# Autodesk Inventor assembly: 2021-2022 Wheel Module
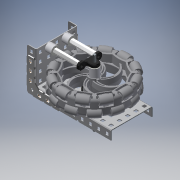
[picture p0: Inventor's stored thumbnail of the model, 180x180]
Saved by Autodesk Inventor 2019 (Build 230136000, 136)
## iProperties
Created: 2021-08-26
Part Number: 2021-2022 Wheel Module
Document SubType Name: Assembly
Designer: 22spencen
Author: 22spencen
## Documents named in this file (13)
- \\Chopper\2022\22spencen\Documents\VEX_CAD\Assemblies\2021-2022 Wheel Module.iam
- U:\Svec\Robotics\Parts\Motion\4_Omni-Directional_Wheel_276-2185.ipt
- U:\Svec\Robotics\Parts\Motion\Metal_Shaft_Inserts_276-3881-002.ipt
- \\Chopper\2022\22spencen\Documents\VEX_CAD\Part Files\VEX Parts Library 2016\Imperial\Structure\C-Channel\C-Channel 1x5x1x10 Hole.ipt
- \\Chopper\2022\22spencen\Documents\VEX_CAD\Part Files\VEX Parts Library 2016\Imperial\Structure\C-Channel 1x5x1x5 Hole.ipt
- \\Chopper\2022\22spencen\Documents\VEX_CAD\Part Files\VEX Parts Library 2016\Imperial\Structure\90 Degree Angle Gusset Outer.ipt
- \\Chopper\2022\22spencen\Documents\VEX_CAD\Part Files\VEX Parts Library 2016\Imperial\Motion\Shafts and Related\Bearing Flat.ipt
- \\Chopper\2022\22spencen\Documents\VEX_CAD\Part Files\VEX Parts Library 2016\Imperial\Motion\Shafts and Related\Shaft 4 inch.ipt
- \\Chopper\2022\22spencen\Documents\VEX_CAD\Part Files\VEX Parts Library 2016\Imperial\Motion\Shafts and Related\Nylon Spacer 0.25 inch.ipt
- \\Chopper\2022\22spencen\Documents\VEX_CAD\Part Files\VEX Parts Library 2016\Imperial\Motion\Shafts and Related\Pillow Block.ipt
- \\Chopper\2022\22spencen\Documents\VEX_CAD\Part Files\VEX Parts Library 2016\Imperial\Structure\Standoffs\1.5 inch Standoff.ipt
- \\Chopper\2022\22spencen\Documents\VEX_CAD\Part Files\VEX Parts Library 2016\Imperial\Motion\Shafts and Related\Nylon Spacer 0.125 inch.ipt
- \\Chopper\2022\22spencen\Documents\VEX_CAD\Part Files\VEX Parts Library 2016\Imperial\Motion\Shafts and Related\Nylon Spacer 0.5 inch.ipt
## Components (19 placed, 12 different names)
1. 4_Omni-Directional_Wheel_276-2185:1 — Mate:17, Mate:18, Mate:19
2. C-Channel 1x5x1x10 Hole:1 — Mate:7, Flush:1, Mate:8, Flush:2, Mate:10, Flush:5, Mate:11, Mate:12, Mate:13
3. C-Channel 1x5x1x5 Hole:1 — Mate:8, Flush:2, Mate:9, Flush:3, Flush:4
4. 90 Degree Angle Gusset Outer:1 — Mate:10, Flush:4, Flush:5
5. 90 Degree Angle Gusset Outer:2 — Mate:7, Flush:1, Mate:9, Flush:3
6. Bearing Flat:1 — Mate:11, Mate:12, Mate:13
7. Metal_Shaft_Inserts_276-3881-002:3 — Mate:17, Mate:18, Mate:19, Mate:22, Insert:1
8. Shaft 4 inch:1 — Mate:26, Mate:27, Mate:28
9. Nylon Spacer 0.25 inch:1 — Mate:22, Insert:1
10. Pillow Block:1 — Insert:2, Insert:3, Insert:8
11. 1.5 inch Standoff:1 — Insert:2, Insert:4
12. 1.5 inch Standoff:2 — Insert:3, Insert:5
13. Nylon Spacer 0.25 inch:2 — Insert:4, Insert:6
14. Nylon Spacer 0.25 inch:3 — Insert:5, Insert:7
15. Nylon Spacer 0.125 inch:1 — Insert:7
16. Nylon Spacer 0.125 inch:2 — Insert:6
17. Nylon Spacer 0.5 inch:1 — Insert:8
18. 4_Omni-Directional_Wheel_276-2185:2 — Mate:23, Mate:24, Mate:25
19. Metal_Shaft_Inserts_276-3881-002:4 — Mate:23, Mate:24, Mate:25, Mate:26, Mate:27, Mate:28
## Relationships (30: Mate 17, Insert 8, Flush 5)
- Mate:7: C-Channel 1x5x1x10 Hole:1 ↔ 90 Degree Angle Gusset Outer:2
- Flush:1: C-Channel 1x5x1x10 Hole:1 ↔ 90 Degree Angle Gusset Outer:2
- Mate:8: C-Channel 1x5x1x10 Hole:1 ↔ C-Channel 1x5x1x5 Hole:1
- Flush:2: C-Channel 1x5x1x10 Hole:1 ↔ C-Channel 1x5x1x5 Hole:1
- Mate:9: C-Channel 1x5x1x5 Hole:1 ↔ 90 Degree Angle Gusset Outer:2
- Flush:3: C-Channel 1x5x1x5 Hole:1 ↔ 90 Degree Angle Gusset Outer:2
- Mate:10: C-Channel 1x5x1x10 Hole:1 ↔ 90 Degree Angle Gusset Outer:1
- Flush:4: C-Channel 1x5x1x5 Hole:1 ↔ 90 Degree Angle Gusset Outer:1
- Flush:5: C-Channel 1x5x1x10 Hole:1 ↔ 90 Degree Angle Gusset Outer:1
- Mate:11: C-Channel 1x5x1x10 Hole:1 ↔ Bearing Flat:1
- Mate:12: C-Channel 1x5x1x10 Hole:1 ↔ Bearing Flat:1
- Mate:13: C-Channel 1x5x1x10 Hole:1 ↔ Bearing Flat:1
- Mate:17: 4_Omni-Directional_Wheel_276-2185:1 ↔ Metal_Shaft_Inserts_276-3881-002:3
- Mate:18: 4_Omni-Directional_Wheel_276-2185:1 ↔ Metal_Shaft_Inserts_276-3881-002:3
- Mate:19: 4_Omni-Directional_Wheel_276-2185:1 ↔ Metal_Shaft_Inserts_276-3881-002:3
- Mate:22: Metal_Shaft_Inserts_276-3881-002:3 ↔ Nylon Spacer 0.25 inch:1
- Insert:1: Metal_Shaft_Inserts_276-3881-002:3 ↔ Nylon Spacer 0.25 inch:1
- Insert:2: Pillow Block:1 ↔ 1.5 inch Standoff:1
- Insert:3: Pillow Block:1 ↔ 1.5 inch Standoff:2
- Insert:4: 1.5 inch Standoff:1 ↔ Nylon Spacer 0.25 inch:2
- Insert:5: 1.5 inch Standoff:2 ↔ Nylon Spacer 0.25 inch:3
- Insert:6: Nylon Spacer 0.25 inch:2 ↔ Nylon Spacer 0.125 inch:2
- Insert:7: Nylon Spacer 0.25 inch:3 ↔ Nylon Spacer 0.125 inch:1
- Insert:8: Pillow Block:1 ↔ Nylon Spacer 0.5 inch:1
- Mate:23: 4_Omni-Directional_Wheel_276-2185:2 ↔ Metal_Shaft_Inserts_276-3881-002:4
- Mate:24: 4_Omni-Directional_Wheel_276-2185:2 ↔ Metal_Shaft_Inserts_276-3881-002:4
- Mate:25: 4_Omni-Directional_Wheel_276-2185:2 ↔ Metal_Shaft_Inserts_276-3881-002:4
- Mate:26: Shaft 4 inch:1 ↔ Metal_Shaft_Inserts_276-3881-002:4
- Mate:27: Shaft 4 inch:1 ↔ Metal_Shaft_Inserts_276-3881-002:4
- Mate:28: Shaft 4 inch:1 ↔ Metal_Shaft_Inserts_276-3881-002:4
